# Autodesk Inventor assembly: ToASI-3
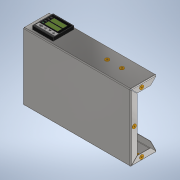
[picture p0: Inventor's stored thumbnail of the model, 180x180]
Saved by Autodesk Inventor 2020.3 (Build 243373000, 373)
## iProperties
Created: 2020-08-01
Part Number: ToASI-3
Document SubType Name: Assembly
Designer: Bruno
Author: Bruno
## Documents named in this file (8)
- C:\Users\Bruno\Desktop\Github\CAD\Inventor\For ASI\ToASI-3.iam
- C:\Users\Bruno\Desktop\Github\CAD\Inventor\For ASI\ToASI-0A.iam
- C:\Users\Bruno\Desktop\Github\CAD\Inventor\Heater-Box\Electric parts\Solid State Rele SSR40DA.ipt
- C:\Users\Bruno\Desktop\Github\CAD\Inventor\Heater-Box\Electric parts\IEC C14 Male panel conector.ipt
- C:\Users\Bruno\Desktop\Github\CAD\Inventor\Heater-Box\Electric parts\DIN7991 M3x0.5x10-8.8 countersunk head cap screws.ipt
- C:\Users\Bruno\Desktop\Github\CAD\Inventor\Heater-Box\Electric parts\DIN934-M3 nut.ipt
- C:\Users\Bruno\Desktop\Github\CAD\Inventor\Heater-Box\Electric parts\Switch OnOff 240V20A.ipt
- C:\Users\Bruno\Desktop\Github\CAD\Inventor\Heater-Box\Electric parts\RexC100 Temp control.ipt
## Components (9 placed, 7 different names)
1. ToASI-0A:1 [sub-assembly] — Mate:1, Mate:2, Mate:3, Cylindrical:1, Slider:1, Slider:2, Mate:4, Mate:5, Mate:6, Rigid:1
2. SSR-XXDA:1 — Mate:1, Mate:2, Mate:3
3. IEC C14 Male panel conector:1 — Cylindrical:1, Cylindrical:3, Cylindrical:4
4. DIN7991 M3x0.5x10-8.8 countersunk head cap screws:1 — Cylindrical:4
5. DIN7991 M3x0.5x10-8.8 countersunk head cap screws:2 — Cylindrical:3
6. DIN934-M3 nut:1 — Slider:1
7. DIN934-M3 nut:2 — Slider:2
8. Switch OnOff 240V20A:1 — Mate:4, Mate:5, Mate:6
9. RexC100 Temp control:1 — Rigid:1
## Relationships (12: Mate 6, CylindricalJoint 3, TranslationJoint 2, WeldJoint 1)
- Mate:1: ToASI-0A:1 ↔ SSR-XXDA:1
- Mate:2 (5 mm): ToASI-0A:1 ↔ SSR-XXDA:1
- Mate:3 (20 mm): ToASI-0A:1 ↔ SSR-XXDA:1
- Cylindrical:1: ToASI-0A:1 ↔ IEC C14 Male panel conector:1
- Cylindrical:3: IEC C14 Male panel conector:1 ↔ DIN7991 M3x0.5x10-8.8 countersunk head cap screws:2
- Cylindrical:4: IEC C14 Male panel conector:1 ↔ DIN7991 M3x0.5x10-8.8 countersunk head cap screws:1
- Slider:1 [TranslationJoint]: ToASI-0A:1 ↔ DIN934-M3 nut:1
- Slider:2 [TranslationJoint]: ToASI-0A:1 ↔ DIN934-M3 nut:2
- Mate:4: ToASI-0A:1 ↔ Switch OnOff 240V20A:1
- Mate:5: ToASI-0A:1 ↔ Switch OnOff 240V20A:1
- Mate:6: ToASI-0A:1 ↔ Switch OnOff 240V20A:1
- Rigid:1 [WeldJoint]: ToASI-0A:1 ↔ RexC100 Temp control:1
